# Autodesk Inventor assembly: Wheel
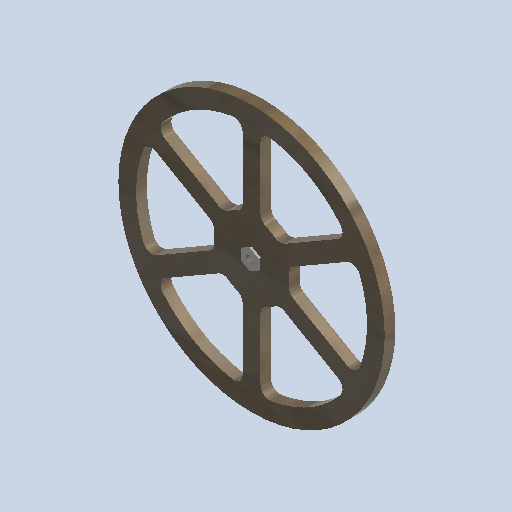
[picture p0: Inventor's stored thumbnail of the model, 512x512]
Saved by Autodesk Inventor 2023 (Build 270158000, 158)
## iProperties
Part Number: Wheel
Document SubType Name: Assembly
Designer: Ronan
Author: Ronan
## Documents named in this file (3)
- D:\Libraries\Documents\2023-FYP\Inventor\Wheel.iam
- D:\Libraries\Documents\2023-FYP\Inventor\wheel.ipt
- D:\Libraries\Documents\2023-FYP\Inventor\Nut-5.ipt
## Components (2 placed, 2 different names)
1. wheel:1 — Mate:1, Mate:2, Flush:1
2. Nut-5:1 — Mate:1, Mate:2, Flush:1
## Relationships (3: Mate 2, Flush 1)
- Mate:1: wheel:1 ↔ Nut-5:1
- Mate:2: wheel:1 ↔ Nut-5:1
- Flush:1: wheel:1 ↔ Nut-5:1
